# Autodesk Inventor assembly: PCBPT_V3
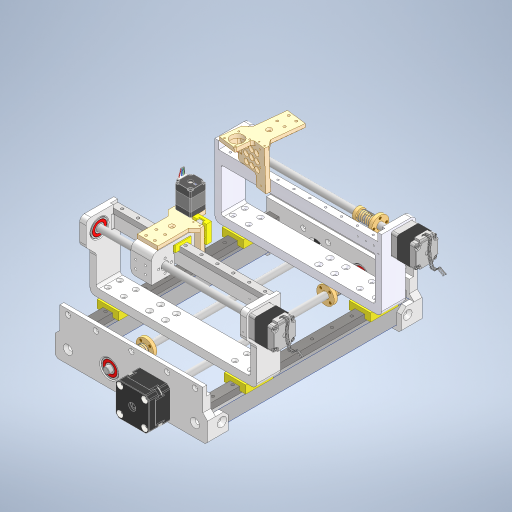
[picture p0: Inventor's stored thumbnail of the model, 512x512]
Saved by Autodesk Inventor 2024.1 (Build 281209000, 209)
## iProperties
Created: 2023-08-11
Part Number: PCBPT_V3
Document SubType Name: Assembly
Designer: l1534
Author: l1534
## Documents named in this file (24)
- C:\DATA\Documents\Lab\github\PCBPT\PCBPT_V3\Mechanical\PCBPT_V3.iam
- C:\DATA\Documents\Lab\github\PCBPT\PCBPT_V3\Mechanical\wall.ipt
- C:\DATA\Documents\Lab\github\PCBPT\PCBPT_V3\Mechanical\NEMA11\NEMA11.iam
- C:\DATA\Documents\Lab\github\PCBPT\PCBPT_V3\Mechanical\2020x260mm.ipt
- C:\DATA\Documents\Lab\github\PCBPT\PCBPT_V3\Mechanical\608-2RS Skate Board Ball Bearing\608-2RS Skate Board Ball Bearing.iam
- C:\DATA\Documents\Lab\github\PCBPT\PCBPT_V3\Mechanical\NEMA_17_PHB42S28-406A v2\NEMA_17_PHB42S28-406A v2.ipt
- C:\DATA\Documents\Lab\github\PCBPT\PCBPT_V3\Mechanical\gantry_R.ipt
- C:\DATA\Documents\Lab\github\PCBPT\PCBPT_V3\Mechanical\gantry_L_MIR.ipt
- C:\DATA\Documents\Lab\github\PCBPT\PCBPT_V3\Mechanical\E_box.ipt
- C:\DATA\Documents\Lab\github\PCBPT\PCBPT_V3\Mechanical\T8x250mm.ipt
- C:\DATA\Documents\Lab\github\PCBPT\PCBPT_V3\Mechanical\T8x200mm.ipt
- C:\DATA\Documents\Lab\github\PCBPT\PCBPT_V3\Mechanical\machine_platform.ipt
- C:\DATA\Documents\Lab\github\FlexiNet\mechanical\V1\MGN12H_rail.ipt
- C:\DATA\Documents\Lab\github\FlexiNet\mechanical\V1\MGN12C_block.ipt
- C:\DATA\Documents\Lab\github\PCBPT\PCBPT_V3\Mechanical\TR8_8(P4) Antibacklash Nut w. spring\TR8_8(P4) Antibacklash Nut w. spring.ipt
- C:\DATA\Documents\Lab\github\PCBPT\PCBPT_V3\Mechanical\probe_block_R.ipt
- C:\DATA\Documents\Lab\github\PCBPT\PCBPT_V3\Mechanical\probe_block_L.ipt
- C:\DATA\Documents\Lab\github\FlexiNet\mechanical\V1\MGN9x200mm_rail.ipt
- C:\DATA\Documents\Lab\github\PCBPT\PCBPT_V3\Mechanical\MGN9C_block.ipt
- C:\DATA\Documents\Lab\github\PCBPT\PCBPT_V3\Mechanical\Motor_holder_R.ipt
- C:\DATA\Documents\Lab\github\PCBPT\PCBPT_V3\Mechanical\SY20STH30-0604A\SY20STH30-0604A.ipt
- C:\DATA\Documents\Lab\github\PCBPT\PCBPT_V3\Mechanical\MGN7c_50mm_rail.ipt
- C:\DATA\Documents\Lab\github\PCBPT\PCBPT_V3\Mechanical\MGN7C_slider.ipt
- C:\DATA\Documents\Lab\github\PCBPT\PCBPT_V3\Mechanical\Motor_holder_L.ipt
## Components (42 placed, 23 different names)
1. wall:1 — Flush:3, Mate:7, Mate:16, Mate:17, Flush:5, Insert:2, Rigid:6
2. 2020x250mm:1 — Rigid:10
3. 2020x250mm:2 — Mate:16, Mate:17, Flush:5, Mate:18, Flush:7, Rigid:11
4. wall:2 — Flush:4, Mate:8, Insert:3
5. 608-2RS Skate Board Ball Bearing:2 [sub-assembly] — Mate:14, Mate:15, Flush:6
6. NEMA_17_PHB42S28-406A v2:1 — Flush:3, Mate:7, Rotational:1
7. NEMA_17_PHB42S28-406A v2:2 — Flush:4, Mate:8, Rotational:2
8. gantry_R:1 — Mate:10, Rigid:8, Rigid:12, Rigid:13, Rigid:19
9. 608-2RS Skate Board Ball Bearing:3 [sub-assembly] — Mate:10
10. gantry_L_MIR:1 — Mate:14, Mate:15, Insert:1, Flush:6, Rigid:14, Rigid:15, Angle:2, Mate:19, Rigid:18
11. NEMA11:6 [sub-assembly] — Insert:1, Rotational:3, Angle:2
12. 608-2RS Skate Board Ball Bearing:4 [sub-assembly] — Insert:2
13. 608-2RS Skate Board Ball Bearing:5 [sub-assembly] — Insert:3
14. E_box:1 — Mate:18, Flush:7
15. T8x250mm:1 — Rotational:1, Cylindrical:4
16. T8x250mm:2 — Rotational:2, Cylindrical:3
17. T8x200mm:1 — Rotational:3, Cylindrical:2
18. T8x200mm:2 — Rotational:4, Cylindrical:1
19. NEMA11:7 [sub-assembly] — Rotational:4, Rigid:8
20. machine_platform:1 — Rigid:6
21. MGN12H_rail:1 — Rigid:10, Slider:7, Slider:8
22. MGN12H_rail:2 — Rigid:11, Slider:9, Slider:10
23. MGN12C_block:1 — Slider:7, Rigid:14
24. MGN12C_block:2 — Slider:8, Rigid:12
25. MGN12C_block:3 — Slider:9, Rigid:15
26. MGN12C_block:4 — Slider:10, Rigid:13
27. TR8_8(P4) Antibacklash Nut w. spring:1 — Cylindrical:1, Rigid:16
28. TR8_8(P4) Antibacklash Nut w. spring:2 — Cylindrical:2, Rigid:17
29. TR8_8(P4) Antibacklash Nut w. spring:3 — Cylindrical:3
30. TR8_8(P4) Antibacklash Nut w. spring:4 — Cylindrical:4
31. probe_block_R:1 — Rigid:16, Mate:22, Rigid:22
32. probe_block_L:1 — Rigid:17, Rigid:20
33. MGN9x200mm_rail:1 — Rigid:19, Mate:21
34. MGN9C_block:1 — Mate:20, Rigid:20
35. MGN9C_block:2 — Mate:21, Mate:22
36. MGN9x200mm_rail:2 — Mate:19, Rigid:18, Mate:20
37. Motor_holder_R:1 — Rigid:21, Rigid:22, Rigid:23
38. SY20STH30-0604A:1 — Rigid:21
39. SY20STH30-0604A:2
40. MGN7c_50mm_rail:1 — Slider:11, Rigid:23
41. MGN7C_slider:1 — Slider:11
42. Motor_holder_L:1
## Relationships (50: WeldJoint 16, Mate 12, Flush 5, TranslationJoint 5, RevoluteJoint 4, CylindricalJoint 4, Insert 3, Angle 1)
- Flush:3: wall:1 ↔ NEMA_17_PHB42S28-406A v2:1
- Flush:4: wall:2 ↔ NEMA_17_PHB42S28-406A v2:2
- Mate:7: wall:1 ↔ NEMA_17_PHB42S28-406A v2:1
- Mate:8: wall:2 ↔ NEMA_17_PHB42S28-406A v2:2
- Mate:10: gantry_R:1 ↔ 608-2RS Skate Board Ball Bearing:3
- Mate:14: 608-2RS Skate Board Ball Bearing:2 ↔ gantry_L_MIR:1
- Mate:15: 608-2RS Skate Board Ball Bearing:2 ↔ gantry_L_MIR:1
- Insert:1: gantry_L_MIR:1 ↔ NEMA11:6
- Mate:16: wall:1 ↔ 2020x250mm:2
- Mate:17: wall:1 ↔ 2020x250mm:2
- Flush:5: wall:1 ↔ 2020x250mm:2
- Insert:2: wall:1 ↔ 608-2RS Skate Board Ball Bearing:4
- Insert:3: wall:2 ↔ 608-2RS Skate Board Ball Bearing:5
- Flush:6: 608-2RS Skate Board Ball Bearing:2 ↔ gantry_L_MIR:1
- Mate:18: 2020x250mm:2 ↔ E_box:1
- Flush:7: 2020x250mm:2 ↔ E_box:1
- Rotational:1 [RevoluteJoint]: NEMA_17_PHB42S28-406A v2:1 ↔ T8x250mm:1
- Rotational:2 [RevoluteJoint]: NEMA_17_PHB42S28-406A v2:2 ↔ T8x250mm:2
- Rotational:3 [RevoluteJoint]: NEMA11:6 ↔ T8x200mm:1
- Rotational:4 [RevoluteJoint]: T8x200mm:2 ↔ NEMA11:7
- Rigid:6 [WeldJoint]: wall:1 ↔ machine_platform:1
- Rigid:8 [WeldJoint]: gantry_R:1 ↔ NEMA11:7
- Rigid:10 [WeldJoint]: 2020x250mm:1 ↔ MGN12H_rail:1
- Rigid:11 [WeldJoint]: 2020x250mm:2 ↔ MGN12H_rail:2
- Slider:7 [TranslationJoint]: MGN12H_rail:1 ↔ MGN12C_block:1
- Slider:8 [TranslationJoint]: MGN12H_rail:1 ↔ MGN12C_block:2
- Slider:9 [TranslationJoint]: MGN12H_rail:2 ↔ MGN12C_block:3
- Slider:10 [TranslationJoint]: MGN12H_rail:2 ↔ MGN12C_block:4
- Rigid:12 [WeldJoint]: gantry_R:1 ↔ MGN12C_block:2
- Rigid:13 [WeldJoint]: gantry_R:1 ↔ MGN12C_block:4
- Rigid:14 [WeldJoint]: gantry_L_MIR:1 ↔ MGN12C_block:1
- Rigid:15 [WeldJoint]: gantry_L_MIR:1 ↔ MGN12C_block:3
- Cylindrical:1: T8x200mm:2 ↔ TR8_8(P4) Antibacklash Nut w. spring:1
- Cylindrical:2: T8x200mm:1 ↔ TR8_8(P4) Antibacklash Nut w. spring:2
- Cylindrical:3: T8x250mm:2 ↔ TR8_8(P4) Antibacklash Nut w. spring:3
- Cylindrical:4: T8x250mm:1 ↔ TR8_8(P4) Antibacklash Nut w. spring:4
- Rigid:16 [WeldJoint]: TR8_8(P4) Antibacklash Nut w. spring:1 ↔ probe_block_R:1
- Angle:2 (0 deg): gantry_L_MIR:1 ↔ NEMA11:6
- Rigid:17 [WeldJoint]: TR8_8(P4) Antibacklash Nut w. spring:2 ↔ probe_block_L:1
- Mate:19: gantry_L_MIR:1 ↔ MGN9x200mm_rail:2
- Rigid:18 [WeldJoint]: gantry_L_MIR:1 ↔ MGN9x200mm_rail:2
- Rigid:19 [WeldJoint]: gantry_R:1 ↔ MGN9x200mm_rail:1
- Mate:20: MGN9C_block:1 ↔ MGN9x200mm_rail:2
- Mate:21: MGN9x200mm_rail:1 ↔ MGN9C_block:2
- Mate:22: probe_block_R:1 ↔ MGN9C_block:2
- Rigid:20 [WeldJoint]: probe_block_L:1 ↔ MGN9C_block:1
- Rigid:21 [WeldJoint]: Motor_holder_R:1 ↔ SY20STH30-0604A:1
- Rigid:22 [WeldJoint]: probe_block_R:1 ↔ Motor_holder_R:1
- Slider:11 [TranslationJoint]: MGN7c_50mm_rail:1 ↔ MGN7C_slider:1
- Rigid:23 [WeldJoint]: Motor_holder_R:1 ↔ MGN7c_50mm_rail:1
